# Autodesk Inventor assembly: PSUMount
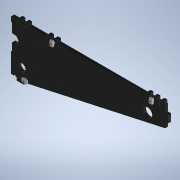
[picture p0: Inventor's stored thumbnail of the model, 180x180]
Saved by Autodesk Inventor 2020.2 (Build 242310000, 310)
## iProperties
Created: 2020-08-24
Part Number: PSUMount
Document SubType Name: Assembly
Designer: JK
Author: JK
## Documents named in this file (4)
- C:\Users\JK\Documents\Inventor\Anet Upgrade\PSUMount.iam
- C:\Users\JK\Documents\Inventor\Anet Upgrade\acrylicframepart.ipt
- C:\Users\JK\Documents\Inventor\Anet Upgrade\T_Slot_Nut_Dropin_3030m5ipt.ipt
- C:\Users\JK\Documents\Inventor\Anet Upgrade\M5x15BoltFlatHead.ipt
## Components (7 placed, 3 different names)
1. acrylicframepart:1 — Mate:1, Mate:2, Mate:3, Angle:1, Mate:7, Mate:8
2. M5x15BoltFlatHead:1 — Mate:1, Mate:6, Mate:7, Flush:1
3. M5x15BoltFlatHead:2 — Mate:2, Mate:4, Flush:1, Flush:2
4. M5x15BoltFlatHead:3 — Mate:3, Mate:5, Flush:2
5. T_Slot_Nut_Dropin_3030m5ipt:1 — Mate:4, Angle:2, Angle:3, Flush:3, Flush:4
6. T_Slot_Nut_Dropin_3030m5ipt:2 — Mate:5, Angle:3, Flush:4
7. T_Slot_Nut_Dropin_3030m5ipt:3 — Mate:6, Angle:1, Angle:2, Mate:8, Flush:3
## Relationships (15: Mate 8, Flush 4, Angle 3)
- Mate:1: acrylicframepart:1 ↔ M5x15BoltFlatHead:1
- Mate:2: acrylicframepart:1 ↔ M5x15BoltFlatHead:2
- Mate:3: acrylicframepart:1 ↔ M5x15BoltFlatHead:3
- Mate:4: M5x15BoltFlatHead:2 ↔ T_Slot_Nut_Dropin_3030m5ipt:1
- Mate:5: M5x15BoltFlatHead:3 ↔ T_Slot_Nut_Dropin_3030m5ipt:2
- Mate:6: M5x15BoltFlatHead:1 ↔ T_Slot_Nut_Dropin_3030m5ipt:3
- Angle:1 (0 deg): acrylicframepart:1 ↔ T_Slot_Nut_Dropin_3030m5ipt:3
- Angle:2 (0 deg): T_Slot_Nut_Dropin_3030m5ipt:1 ↔ T_Slot_Nut_Dropin_3030m5ipt:3
- Angle:3 (90 deg): T_Slot_Nut_Dropin_3030m5ipt:1 ↔ T_Slot_Nut_Dropin_3030m5ipt:2
- Mate:7: acrylicframepart:1 ↔ M5x15BoltFlatHead:1
- Flush:1: M5x15BoltFlatHead:1 ↔ M5x15BoltFlatHead:2
- Flush:2: M5x15BoltFlatHead:2 ↔ M5x15BoltFlatHead:3
- Mate:8: acrylicframepart:1 ↔ T_Slot_Nut_Dropin_3030m5ipt:3
- Flush:3: T_Slot_Nut_Dropin_3030m5ipt:1 ↔ T_Slot_Nut_Dropin_3030m5ipt:3
- Flush:4: T_Slot_Nut_Dropin_3030m5ipt:1 ↔ T_Slot_Nut_Dropin_3030m5ipt:2
